# Autodesk Inventor assembly: 2inDome
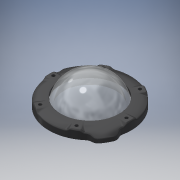
[picture p0: Inventor's stored thumbnail of the model, 180x180]
Saved by Autodesk Inventor 2018 (Build 220112000, 112)
## iProperties
Created: 2019-02-19
Part Number: 2inDome
Description: STEP AP214
Document SubType Name: Assembly
Designer: anirudh
Title: WTE2-ASM-DOME-R1.STEP
Revision Number: ANY
## Documents named in this file (3)
- C:\Users\anirudh\Documents\MARS Fund\MATE Robotics\Silicon Sharks\2018-2019\Prototype3\Dome(2in)\2inDome.iam
- C:\Users\anirudh\Documents\MARS Fund\MATE Robotics\Silicon Sharks\2018-2019\Prototype3\Dome(2in)\WTE2-P-DOME-R1.ipt
- C:\Users\anirudh\Documents\MARS Fund\MATE Robotics\Silicon Sharks\2018-2019\Prototype3\Dome(2in)\WTE2-P-RETAINING-RING-R1.ipt
## Components (2 placed, 2 different names)
1. WTE2-P-DOME-R1_1 — Mate:1
2. WTE2-P-RETAINING-RING-R1_2
## Relationships (1: Mate 1)
- Mate:1: WTE2-P-DOME-R1_1
